# Autodesk Inventor assembly: motor
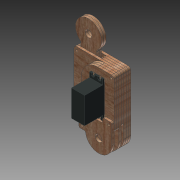
[picture p0: Inventor's stored thumbnail of the model, 180x180]
Saved by Autodesk Inventor 2015 (Build 190159000, 159)
## iProperties
Created: 2016-02-03
Part Number: motor
Document SubType Name: Assembly
Designer: david
Author: david
## Documents named in this file (12)
- Z:\gip\Inventor\generatie 7\Motor\Motor.iam
- Z:\gip\Inventor\generatie 7\Motor\p1.ipt
- Z:\gip\Inventor\generatie 7\Motor\p2.ipt
- Z:\gip\Inventor\generatie 7\Motor\p3.ipt
- Z:\gip\Inventor\generatie 7\Motor\servo\tang.ipt
- Z:\gip\Inventor\generatie 7\Motor\p4.ipt
- Z:\gip\Inventor\generatie 7\Motor\p5.ipt
- Z:\gip\Inventor\generatie 7\Motor\servo\block.ipt
- Z:\gip\Inventor\generatie 7\old\Motor\tanden.ipt
- Z:\gip\Inventor\generatie 7\Motor\tandwiel\tandwiel.iam
- Z:\gip\Inventor\generatie 7\Motor\p6.ipt
- Z:\gip\Inventor\generatie 7\Motor\p5 - big.ipt
## Components (13 placed, 11 different names)
1. p1:1 — Mate:1, Flush:1, Flush:2, Flush:4
2. p2:1 — Mate:1, Flush:1, Flush:2, Mate:2, Flush:3, Flush:5
3. p2:2 — Mate:2, Flush:3, Flush:4, Mate:3, Flush:6, Mate:14, Mate:15, Mate:21
4. p3:1 — Mate:3, Flush:5, Flush:6, Flush:7, Flush:8, Mate:5, Mate:13
5. p4:1 — Flush:7, Flush:8, Mate:5, Flush:9, Flush:10, Mate:6
6. p5 - big:1 — Flush:9, Flush:10, Mate:6, Flush:11, Flush:12, Mate:7, Mate:17
7. p5:2 — Flush:11, Flush:12, Mate:7, Mate:8, Mate:9, Mate:12, Flush:14
8. block:1 — Mate:8, Mate:9, Mate:10, Mate:11, Mate:12
9. tang:1 — Mate:10, Mate:11, Mate:16, Mate:18
10. tanden:1 — Mate:13, Mate:14, Mate:15, Rotation/Translation:1, Mate:19, Flush:13, Mate:20
11. tandwiel:1 [sub-assembly] — Mate:16, Mate:17, Mate:18, Rotation/Translation:1
12. tanden:2 — Mate:19, Flush:13, Mate:20, Mate:21
13. p6:1 — Flush:14
## Relationships (35: Mate 20, Flush 14, RelateRotateTranslate 1)
- Mate:1: p1:1 ↔ p2:1
- Flush:1: p1:1 ↔ p2:1
- Flush:2: p1:1 ↔ p2:1
- Mate:2: p2:1 ↔ p2:2
- Flush:3: p2:1 ↔ p2:2
- Flush:4: p1:1 ↔ p2:2
- Mate:3: p2:2 ↔ p3:1
- Flush:5: p2:1 ↔ p3:1
- Flush:6: p2:2 ↔ p3:1
- Flush:7: p3:1 ↔ p4:1
- Flush:8: p3:1 ↔ p4:1
- Mate:5: p3:1 ↔ p4:1
- Flush:9: p4:1 ↔ p5 - big:1
- Flush:10: p4:1 ↔ p5 - big:1
- Mate:6: p4:1 ↔ p5 - big:1
- Flush:11: p5 - big:1 ↔ p5:2
- Flush:12: p5 - big:1 ↔ p5:2
- Mate:7: p5 - big:1 ↔ p5:2
- Mate:8: p5:2 ↔ block:1
- Mate:9: p5:2 ↔ block:1
- Mate:10: block:1 ↔ tang:1
- Mate:11: block:1 ↔ tang:1
- Mate:12: p5:2 ↔ block:1
- Mate:13: p3:1 ↔ tanden:1
- Mate:14: p2:2 ↔ tanden:1
- Mate:15: p2:2 ↔ tanden:1
- Mate:16 (0.15 mm): tang:1 ↔ tandwiel:1
- Mate:17: p5 - big:1 ↔ tandwiel:1
- Mate:18: tang:1 ↔ tandwiel:1
- Rotation/Translation:1 [RelateRotateTranslate] (100 mm): tanden:1 ↔ tandwiel:1
- Mate:19: tanden:1 ↔ tanden:2
- Flush:13: tanden:1 ↔ tanden:2
- Mate:20: tanden:1 ↔ tanden:2
- Flush:14: p5:2 ↔ p6:1
- Mate:21: p2:2 ↔ tanden:2
